# Autodesk Inventor assembly: HB8_900.1-sunhub8-casing
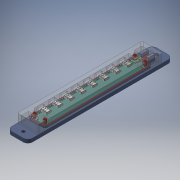
[picture p0: Inventor's stored thumbnail of the model, 180x180]
Saved by Autodesk Inventor 2019 (Build 230136000, 136)
## iProperties
Created: 2019-02-22
Part Number: HB8_900.1-sunhub8-casing
Document SubType Name: Assembly
Designer: Rene
Author: Rene
## Documents named in this file (5)
- C:\dev\c-scape\hardponics\dwg\sunhub\HB8_900.1-sunhub8-casing.iam
- C:\dev\c-scape\hardponics\dwg\sunhub\SH8_001.1-sunhub8-casing_bottom.ipt
- C:\dev\c-scape\hardponics\dwg\sunhub\XGEN_M3_screw.ipt
- C:\dev\c-scape\hardponics\dwg\sunhub\HB8_910.1-sunhub8_pcb.iam
- C:\dev\c-scape\hardponics\dwg\sunhub\HB8_920.1-sunhub8_casing_top.iam
## Components (7 placed, 4 different names)
1. SH8_001.1-sunhub8-casing_bottom:1 — Insert:1, Insert:2, Insert:3, Insert:4, Mate:8
2. HB8_910.1-sunhub8_pcb:1 [sub-assembly] — Mate:6, Mate:7, Mate:8
3. XGEN_M3_screw:1 — Insert:1
4. XGEN_M3_screw:2 — Insert:2, Mate:6, Mate:9
5. XGEN_M3_screw:3 — Insert:3, Mate:7, Mate:10
6. XGEN_M3_screw:4 — Insert:4
7. HB8_920.1-sunhub8_casing_top:1 [sub-assembly] — Mate:9, Mate:10
## Relationships (9: Mate 5, Insert 4)
- Insert:1: SH8_001.1-sunhub8-casing_bottom:1 ↔ XGEN_M3_screw:1
- Insert:2: SH8_001.1-sunhub8-casing_bottom:1 ↔ XGEN_M3_screw:2
- Insert:3: SH8_001.1-sunhub8-casing_bottom:1 ↔ XGEN_M3_screw:3
- Insert:4: SH8_001.1-sunhub8-casing_bottom:1 ↔ XGEN_M3_screw:4
- Mate:6: HB8_910.1-sunhub8_pcb:1 ↔ XGEN_M3_screw:2
- Mate:7: HB8_910.1-sunhub8_pcb:1 ↔ XGEN_M3_screw:3
- Mate:8: SH8_001.1-sunhub8-casing_bottom:1 ↔ HB8_910.1-sunhub8_pcb:1
- Mate:9: XGEN_M3_screw:2 ↔ HB8_920.1-sunhub8_casing_top:1
- Mate:10: XGEN_M3_screw:3 ↔ HB8_920.1-sunhub8_casing_top:1
